# Autodesk Inventor assembly: Gehäuse
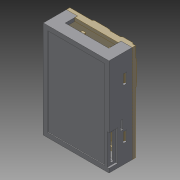
[picture p0: Inventor's stored thumbnail of the model, 180x180]
Saved by Autodesk Inventor 2014 (Build 180170000, 170)
## iProperties
Created: 2016-07-27
Part Number: Gehäuse
Document SubType Name: Assembly
Designer: cem
Author: cem
## Documents named in this file (4)
- C:\development\AnySense\Hardware\Gehäuse\Gehäuse.iam
- C:\development\AnySense\Hardware\Gehäuse\Platine.ipt
- C:\development\AnySense\Hardware\Gehäuse\Boden.ipt
- C:\development\AnySense\Hardware\Gehäuse\Deckel.ipt
## Components (3 placed, 3 different names)
1. Platine:1 — Fluchtend:1, Fluchtend:2, Fluchtend:3, Fluchtend:12, Fluchtend:13
2. Boden:1 — Fluchtend:1, Fluchtend:2, Fluchtend:3, Fluchtend:4, Fluchtend:5, Fluchtend:7, Fluchtend:14
3. Deckel:1 — Fluchtend:4, Fluchtend:5, Fluchtend:7, Fluchtend:12, Fluchtend:13, Fluchtend:14
## Relationships (9: Flush 9)
- Fluchtend:1 [Flush]: Platine:1 ↔ Boden:1
- Fluchtend:2 [Flush] (0.05 mm): Platine:1 ↔ Boden:1
- Fluchtend:3 [Flush] (1.5 mm): Platine:1 ↔ Boden:1
- Fluchtend:4 [Flush]: Boden:1 ↔ Deckel:1
- Fluchtend:5 [Flush] (0.05 mm): Boden:1 ↔ Deckel:1
- Fluchtend:7 [Flush] (0.15 mm): Boden:1 ↔ Deckel:1
- Fluchtend:12 [Flush] (0.3 mm): Platine:1 ↔ Deckel:1
- Fluchtend:13 [Flush] (0.05 mm): Platine:1 ↔ Deckel:1
- Fluchtend:14 [Flush] (-0.8 mm): Boden:1 ↔ Deckel:1
